# Autodesk Inventor assembly: Drivetrain Encoder Sprocket
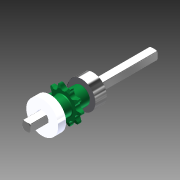
[picture p0: Inventor's stored thumbnail of the model, 180x180]
Saved by Autodesk Inventor 2012 (Build 160160000, 160)
## iProperties
Created: 2011-09-12
Part Number: Drivetrain Encoder Sprocket
Document SubType Name: Assembly
Designer: Wade
Author: Wade
## Documents named in this file (5)
- C:\Users\Wade\Documents\1103 Robot - CAD Assembly\Drivetrain Encoder Sprocket.iam
- C:\Users\Wade\Documents\24C VEX CAD Files\Drive Shafts\Drive Shaft (Square Bar) 2''.ipt
- C:\Users\Wade\Documents\24C VEX CAD Files\Gears & Pulleys\10-Tooth Sprocket.ipt
- C:\Users\Wade\Documents\24C VEX CAD Files\Washers & Spacers\Spacer (Nylon), 0.125''.ipt
- C:\Users\Wade\Documents\24C VEX CAD Files\Other Parts\Shaft Collar (thin).ipt
## Components (4 placed, 4 different names)
1. Drive Shaft (Square Bar) 2'':1 — Mate:1, Mate:2, Flush:1, Flush:2
2. 10-Tooth Sprocket:1 — Mate:1, Mate:2, Flush:1, Mate:3, Mate:4, Mate:5, Mate:6
3. Spacer (Nylon), 0.125'':1 — Mate:3, Mate:4
4. Shaft Collar (thin):1 — Mate:5, Mate:6, Flush:2
## Relationships (8: Mate 6, Flush 2)
- Mate:1: Drive Shaft (Square Bar) 2'':1 ↔ 10-Tooth Sprocket:1
- Mate:2: Drive Shaft (Square Bar) 2'':1 ↔ 10-Tooth Sprocket:1
- Flush:1 (9.525 mm): Drive Shaft (Square Bar) 2'':1 ↔ 10-Tooth Sprocket:1
- Mate:3: 10-Tooth Sprocket:1 ↔ Spacer (Nylon), 0.125'':1
- Mate:4: 10-Tooth Sprocket:1 ↔ Spacer (Nylon), 0.125'':1
- Mate:5: 10-Tooth Sprocket:1 ↔ Shaft Collar (thin):1
- Mate:6: 10-Tooth Sprocket:1 ↔ Shaft Collar (thin):1
- Flush:2: Drive Shaft (Square Bar) 2'':1 ↔ Shaft Collar (thin):1
